# Autodesk Inventor assembly: Crabot 1-4 to 11-32
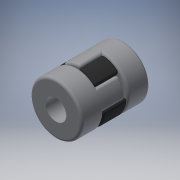
[picture p0: Inventor's stored thumbnail of the model, 180x180]
Saved by Autodesk Inventor 2018 (Build 220112000, 112)
## iProperties
Created: 2020-03-23
Part Number: Crabot 1-4 to 11-32
Document SubType Name: Assembly
Designer: emile
Author: emile
## Documents named in this file (4)
- C:\Users\emile\OneDrive\Documents\Inventor\Respirator\Crabot 1-4 to 11-32.iam
- C:\Users\emile\OneDrive\Documents\Inventor\Respirator\Flexible Shaft Coupling Iron Hub 1-4.ipt
- C:\Users\emile\OneDrive\Documents\Inventor\Respirator\Flexible Shaft Coupling Iron Hub 11-32.ipt
- C:\Users\emile\OneDrive\Documents\Inventor\Respirator\crabot.ipt
## Components (3 placed, 3 different names)
1. Flexible Shaft Coupling Iron Hub 1-4:1 — Mate:1, Mate:2, Mate:7, Mate:9
2. Flexible Shaft Coupling Iron Hub 11-32:1 — Mate:1, Mate:2, Mate:3, Mate:4, Mate:5, Mate:6, Mate:8
3. crabot:1 — Mate:7, Mate:8, Mate:9
## Relationships (9: Mate 9)
- Mate:1: Flexible Shaft Coupling Iron Hub 1-4:1 ↔ Flexible Shaft Coupling Iron Hub 11-32:1
- Mate:2 (0.7112 mm): Flexible Shaft Coupling Iron Hub 1-4:1 ↔ Flexible Shaft Coupling Iron Hub 11-32:1
- Mate:3: Flexible Shaft Coupling Iron Hub 11-32:1
- Mate:4: Flexible Shaft Coupling Iron Hub 11-32:1
- Mate:5: Flexible Shaft Coupling Iron Hub 11-32:1
- Mate:6: Flexible Shaft Coupling Iron Hub 11-32:1
- Mate:7: Flexible Shaft Coupling Iron Hub 1-4:1 ↔ crabot:1
- Mate:8: Flexible Shaft Coupling Iron Hub 11-32:1 ↔ crabot:1
- Mate:9: Flexible Shaft Coupling Iron Hub 1-4:1 ↔ crabot:1
